# Autodesk Inventor assembly: Assembly
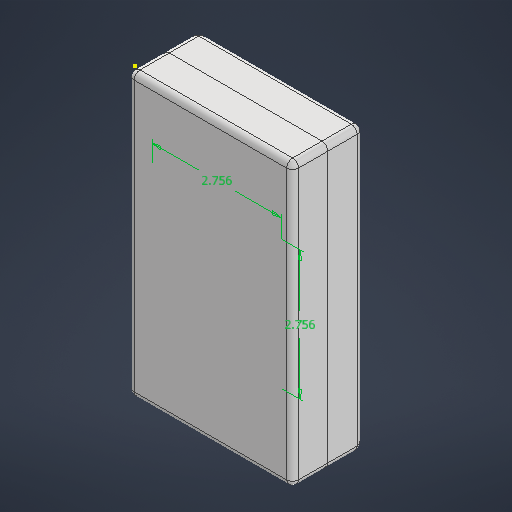
[picture p0: Inventor's stored thumbnail of the model, 512x512]
Saved by Autodesk Inventor 2026.2 (Build 302298010, 298A)
## iProperties
Created: 2026-03-08
Part Number: Assembly
Document SubType Name: Assembly
Designer: kjedr
Author: kjedr
## Documents named in this file (4)
- C:\Users\kjedr\Documents\Autodesk\Assembly.iam
- C:\Users\kjedr\Documents\Autodesk\Top_Shell.ipt
- C:\Users\kjedr\Documents\Autodesk\Bottom_Shell.ipt
- C:\Users\kjedr\Documents\Autodesk\Dial.ipt
## Components (3 placed, 3 different names)
1. Top_Shell:1 — Mate:1, Flush:1, Flush:2, Insert:1
2. Bottom_Shell:1 — Mate:1, Flush:1, Flush:2
3. Dial:1 — Insert:1
## Relationships (4: Flush 2, Mate 1, Insert 1)
- Mate:1: Top_Shell:1 ↔ Bottom_Shell:1
- Flush:1: Top_Shell:1 ↔ Bottom_Shell:1
- Flush:2: Top_Shell:1 ↔ Bottom_Shell:1
- Insert:1: Top_Shell:1 ↔ Dial:1
